# Autodesk Inventor assembly: dads trunk assembly
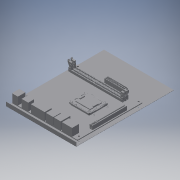
[picture p0: Inventor's stored thumbnail of the model, 180x180]
Saved by Autodesk Inventor 2018 (Build 220112000, 112)
## iProperties
Created: 2018-06-19
Part Number: dads trunk assembly
Document SubType Name: Assembly
Designer: John Viljoen
Author: John Viljoen
## Documents named in this file (3)
- C:\Users\John Viljoen\Documents\Inventor\computer project\dads trunk assembly.iam
- C:\Users\John Viljoen\Documents\Inventor\computer project\dads trunk.ipt
- C:\Users\John Viljoen\Documents\Inventor\computer project\Mini-ITX Mobo.ipt
## Components (2 placed, 2 different names)
1. dads trunk:1 — Mate:1, Flush:1, Flush:2
2. Mini-ITX Mobo:1 — Mate:1, Flush:1, Flush:2
## Relationships (3: Flush 2, Mate 1)
- Mate:1 (11 mm): dads trunk:1 ↔ Mini-ITX Mobo:1
- Flush:1: dads trunk:1 ↔ Mini-ITX Mobo:1
- Flush:2 (3.82 mm): dads trunk:1 ↔ Mini-ITX Mobo:1
